# Autodesk Inventor assembly: LoadCellAssembly
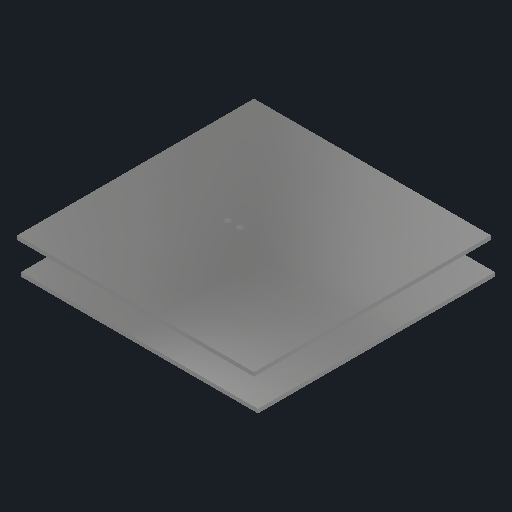
[picture p0: Inventor's stored thumbnail of the model, 512x512]
Saved by Autodesk Inventor 2027 (Build 310192060, 192F)
## iProperties
Created: 2026-09-27
Part Number: LoadCellAssembly
Document SubType Name: Assembly
Designer: notra
Author: notra
## Documents named in this file (3)
- C:\Users\notra\Documents\Pedro\SBESC\Model3D\LoadCellAssembly.iam
- C:\Users\notra\Documents\Pedro\SBESC\Model3D\PlataformaLoadCell.ipt
- C:\Users\notra\Documents\Pedro\SBESC\Model3D\Loadcell_straight_bar_10kg_20Kg\Loadcell_straight_bar_10kg_20Kg.iam
## Components (3 placed, 2 different names)
1. PlataformaLoadCell:1 — Mate:1, Mate:2, Mate:3
2. PlataformaLoadCell:2 — Mate:4, Mate:5, Mate:6
3. Loadcell_straight_bar_10kg_20Kg:1 [sub-assembly] — Mate:1, Mate:2, Mate:3, Mate:4, Mate:5, Mate:6
## Relationships (6: Mate 6)
- Mate:1: PlataformaLoadCell:1 ↔ Loadcell_straight_bar_10kg_20Kg:1
- Mate:2: PlataformaLoadCell:1 ↔ Loadcell_straight_bar_10kg_20Kg:1
- Mate:3: PlataformaLoadCell:1 ↔ Loadcell_straight_bar_10kg_20Kg:1
- Mate:4: PlataformaLoadCell:2 ↔ Loadcell_straight_bar_10kg_20Kg:1
- Mate:5: PlataformaLoadCell:2 ↔ Loadcell_straight_bar_10kg_20Kg:1
- Mate:6: PlataformaLoadCell:2 ↔ Loadcell_straight_bar_10kg_20Kg:1
